# Autodesk Inventor assembly: 100-10-FRAME-BOTTOM-PLATE
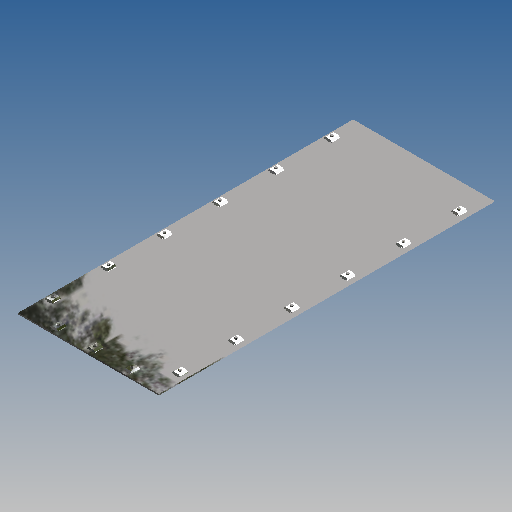
[picture p0: Inventor's stored thumbnail of the model, 512x512]
Saved by Autodesk Inventor 2018.2 (Build 222227000, 227)
## iProperties
Manager: feesmrt
Company: FRANCOR
Part Number: 100-10-FRAME-BOTTOM-PLATE
Project: Rescue Robot
Cost Center: -
Material: Generisch
Document SubType Name: Assembly
Designer: feesmrt
Engineer: feesmrt
Authority: feesmrt
Subject: Rescue Robot
Author: feesmrt
Revision Number: 1
## Documents named in this file (5)
- C:\Users\feesmrt\Documents\FRANC0R\CAD\02-Rocker-Bogie-Robot\100-CHASSIS\10-FRAME\100-10-FRAME-BOTTOM-PLATE.iam
- C:\Users\feesmrt\Documents\FRANC0R\CAD\02-Rocker-Bogie-Robot\100-CHASSIS\10-FRAME\100-10-FRAME-BOTTOM-PLATE.ipt
- C:\Users\feesmrt\Documents\FRANC0R\CAD\02-Rocker-Bogie-Robot\900-COMPONENTS\900-50-PROFILES\900-50-PROFILES-CONN-N6xM4.ipt
- C:\Users\feesmrt\Documents\FRANC0R\CAD\02-Rocker-Bogie-Robot\900-COMPONENTS\900-40-SCREWS\900-40-SCREWS-ISO7830_M4x8.ipt
- C:\Users\feesmrt\Documents\FRANC0R\CAD\02-Rocker-Bogie-Robot\100-CHASSIS\Chassis-Dimensions.xlsx
## Components (31 placed, 3 different names)
1. 100-10-FRAME-BOTTOM-PLATE:1 — Passend:2, Winkel:1, Passend:4, Passend:5, Passend:6, Passend:7, Passend:9, Winkel:2
2. 900-50-PROFILES-CONN-N6xM4:1 — Passend:2, Winkel:1, Passend:3
3. 900-40-SCREWS-ISO7830_M4x8:1 — Passend:3, Passend:4, Passend:5
4. 900-50-PROFILES-CONN-N6xM4:2
5. 900-40-SCREWS-ISO7830_M4x8:2
6. 900-50-PROFILES-CONN-N6xM4:3
7. 900-40-SCREWS-ISO7830_M4x8:3
8. 900-50-PROFILES-CONN-N6xM4:4
9. 900-40-SCREWS-ISO7830_M4x8:4
10. 900-50-PROFILES-CONN-N6xM4:5
11. 900-40-SCREWS-ISO7830_M4x8:5
12. 900-50-PROFILES-CONN-N6xM4:6
13. 900-40-SCREWS-ISO7830_M4x8:6
14. 900-50-PROFILES-CONN-N6xM4:7
15. 900-40-SCREWS-ISO7830_M4x8:7
16. 900-50-PROFILES-CONN-N6xM4:8
17. 900-40-SCREWS-ISO7830_M4x8:8
18. 900-50-PROFILES-CONN-N6xM4:9
19. 900-40-SCREWS-ISO7830_M4x8:9
20. 900-50-PROFILES-CONN-N6xM4:10
21. 900-40-SCREWS-ISO7830_M4x8:10
22. 900-50-PROFILES-CONN-N6xM4:11
23. 900-40-SCREWS-ISO7830_M4x8:11
24. 900-50-PROFILES-CONN-N6xM4:12
25. 900-40-SCREWS-ISO7830_M4x8:12
26. 900-40-SCREWS-ISO7830_M4x8:21 — Passend:6, Passend:7, Passend:8
27. 900-50-PROFILES-CONN-N6xM4:21 — Passend:8, Passend:9, Winkel:2
28. 900-40-SCREWS-ISO7830_M4x8:22
29. 900-50-PROFILES-CONN-N6xM4:22
30. 900-40-SCREWS-ISO7830_M4x8:23
31. 900-50-PROFILES-CONN-N6xM4:23
## Component patterns: (12 elements, first: 900-50-PROFILES-CONN-N6xM4:1 + 900-40-SCREWS-ISO7830_M4x8:1), (3 elements, first: 900-40-SCREWS-ISO7830_M4x8:21 + 900-50-PROFILES-CONN-N6xM4:21)
## Relationships (10: Mate 8, Angle 2)
- Passend:2 [Mate] (1.5 mm): 100-10-FRAME-BOTTOM-PLATE:1 ↔ 900-50-PROFILES-CONN-N6xM4:1
- Winkel:1 [Angle] (0 deg): 100-10-FRAME-BOTTOM-PLATE:1 ↔ 900-50-PROFILES-CONN-N6xM4:1
- Passend:3 [Mate]: 900-50-PROFILES-CONN-N6xM4:1 ↔ 900-40-SCREWS-ISO7830_M4x8:1
- Passend:4 [Mate]: 100-10-FRAME-BOTTOM-PLATE:1 ↔ 900-40-SCREWS-ISO7830_M4x8:1
- Passend:5 [Mate]: 100-10-FRAME-BOTTOM-PLATE:1 ↔ 900-40-SCREWS-ISO7830_M4x8:1
- Passend:6 [Mate]: 100-10-FRAME-BOTTOM-PLATE:1 ↔ 900-40-SCREWS-ISO7830_M4x8:21
- Passend:7 [Mate]: 100-10-FRAME-BOTTOM-PLATE:1 ↔ 900-40-SCREWS-ISO7830_M4x8:21
- Passend:8 [Mate]: 900-40-SCREWS-ISO7830_M4x8:21 ↔ 900-50-PROFILES-CONN-N6xM4:21
- Passend:9 [Mate] (1.5 mm): 100-10-FRAME-BOTTOM-PLATE:1 ↔ 900-50-PROFILES-CONN-N6xM4:21
- Winkel:2 [Angle] (0 deg): 100-10-FRAME-BOTTOM-PLATE:1 ↔ 900-50-PROFILES-CONN-N6xM4:21
## Named parameters: Chassis_Frame_Size = 30 mm, Chassis_Length = 500 mm, Chassis_Width = 220 mm, Rocker_Bearing_Size = 100 mm, Rocker_Screw_Distance = 32.5 mm, Rocker_Screw_Distance_Bottom = 76 mm, Chassis_Bottom_Height = 80 mm
